# Autodesk Inventor assembly: CNC-FullAssembly
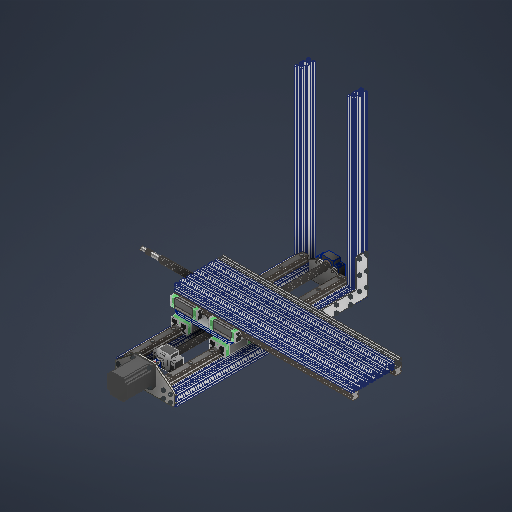
[picture p0: Inventor's stored thumbnail of the model, 512x512]
Saved by Autodesk Inventor 2026.2 (Build 302298000, 298)
## iProperties
Created: 2026-06-14
Part Number: CNC-FullAssembly
Document SubType Name: Assembly
Designer: Kenji
Mass: 13300 g
Surface Area: 16623.1 cm^2
Volume: 2793.26 cm^3
Density: 4.76145 g/cm^3
Author: Kenji
## Documents named in this file (29)
- C:\Users\Kenji\Documents\GitHub\DiyCNC-\CNC-FullAssembly.iam
- C:\Users\Kenji\Documents\GitHub\DiyCNC-\COTS-Parts\40x40x500mm-Extrusion.ipt
- C:\Users\Kenji\Documents\GitHub\DiyCNC-\COTS-Parts\SFU1605-BallScrewNut.iam
- C:\Users\Kenji\Documents\GitHub\DiyCNC-\COTS-Parts\DSG16H-BallScrewFixtureBlock.ipt
- C:\Users\Kenji\Documents\GitHub\DiyCNC-\COTS-Parts\SFU1605-BallScrew500mm.ipt
- C:\Users\Kenji\Documents\GitHub\DiyCNC-\COTS-Parts\BK12-BallScrewStabilizer.iam
- C:\Users\Kenji\Documents\GitHub\DiyCNC-\COTS-Parts\HGR20R-LinearRail500mm.ipt
- C:\Users\Kenji\Documents\GitHub\DiyCNC-\COTS-Parts\HGH20-LinearRailCarriage.iam
- C:\Users\Kenji\Documents\GitHub\DiyCNC-\COTS-Parts\91274A131_M5x20mm.ipt
- C:\Users\Kenji\Documents\GitHub\DiyCNC-\COTS-Parts\91290A231-M5x15mm.ipt
- C:\Users\Kenji\Documents\GitHub\DiyCNC-\COTS-Parts\Nema23-StepperMotor.ipt
- C:\Users\Kenji\Documents\GitHub\DiyCNC-\COTS-Parts\MH2025-6.35x10mmCoupler.iam
- C:\Users\Kenji\Documents\GitHub\DiyCNC-\COTS-Parts\BF12-BallScrewStabilizer2.ipt
- C:\Users\Kenji\Documents\GitHub\DiyCNC-\CNC-000-StructureGusset1.ipt
- C:\Users\Kenji\Documents\GitHub\DiyCNC-\COTS-Parts\20x40x500mm-Extrusion.ipt
- C:\Users\Kenji\Documents\GitHub\DiyCNC-\CNC-001-StructureGusset2.ipt
- C:\Users\Kenji\Documents\GitHub\DiyCNC-\CNC-002-ShimStructureGusset2.ipt
- C:\Users\Kenji\Documents\GitHub\DiyCNC-\COTS-Parts\90576A104-M5-NylockNut.ipt
- C:\Users\Kenji\Documents\GitHub\DiyCNC-\COTS-Parts\91292A195-M5x45mm.ipt
- C:\Users\Kenji\Documents\GitHub\DiyCNC-\CNC-003-StructureGusset3.ipt
- C:\Users\Kenji\Documents\GitHub\DiyCNC-\CNC-004-Nema23Shim.ipt
- C:\Users\Kenji\Documents\GitHub\DiyCNC-\COTS-Parts\91274A125-M5x8mm.ipt
- C:\Users\Kenji\Documents\GitHub\DiyCNC-\CNC-005-XAxisMount1.ipt
- C:\Users\Kenji\Documents\GitHub\DiyCNC-\COTS-Parts\91263A832-M5x10mm-Countersink.ipt
- C:\Users\Kenji\Documents\GitHub\DiyCNC-\CNC-006-XAxisMount2.ipt
- C:\Users\Kenji\Documents\GitHub\DiyCNC-\COTS-Parts\92095A495-M8-18mm-ButtonHead.ipt
- C:\Users\Kenji\Documents\GitHub\DiyCNC-\COTS-Parts\94645A210-M8-NylockNut.ipt
- C:\Users\Kenji\Documents\GitHub\DiyCNC-\COTS-Parts\20x40x500mm-Extrusion2.ipt
- C:\Users\Kenji\Documents\GitHub\DiyCNC-\COTS-Parts\20x20x500mm_Extrusion.ipt
## Components (172 placed, 28 different names)
1. 40x40x500mm-Extrusion:1 — Mate:1, Mate:2, Flush:1, Flush:2, Flush:3, Angle:1, Mate:6, Mate:12, Flush:5, Flush:6, Angle:3, Angle:4, Mate:46, Flush:20, Flush:21, Mate:48, Mate:49, Mate:50, Flush:35
2. 40x40x500mm-Extrusion:2 — Flush:2, Flush:3, Mate:7, Angle:2, Mate:11, Flush:9, Mate:39, Mate:40, Mate:41, Flush:22, Mate:47, Flush:23, Flush:38
3. SFU1605-BallScrewNut:1 [sub-assembly] — Mate:3, Mate:4, Mate:5, Mate:8, Mate:21, Mate:22, Mate:23, Mate:24, Mate:25, Mate:26, Mate:27
4. DSG16H-BallScrewFixtureBlock:1 — Mate:3, Mate:4, Mate:5, Angle:1, Mate:6, Mate:7, Flush:14, Mate:20, Rotation/Translation:2, Angle:6, Mate:98, Mate:99
5. SFU1605-BallScrew500mm:1 — Mate:8, Mate:9, Mate:10, Mate:30, Mate:34, Mate:35, Mate:36, Rotation/Translation:2
6. BK12-BallScrewStabilizer:1 [sub-assembly] — Mate:9, Mate:10, Angle:2
7. HGR20R-LinearRail500mm:1 — Mate:12, Flush:5, Flush:6, Flush:7, Flush:8, Mate:13, Mate:14, Mate:17, Mate:28, Mate:29, Mate:37
8. HGR20R-LinearRail500mm:2 — Mate:11, Flush:7, Flush:8, Flush:9, Mate:15, Mate:16, Mate:19
9. HGH20-LinearRailCarriage:1 [sub-assembly] — Mate:13, Mate:14, Flush:10, Flush:11, Mate:18, Flush:14, Mate:100
10. HGH20-LinearRailCarriage:2 [sub-assembly] — Mate:19, Flush:12, Flush:13
11. HGH20-LinearRailCarriage:3 [sub-assembly] — Mate:15, Mate:16, Flush:10, Flush:12, Mate:20
12. HGH20-LinearRailCarriage:4 [sub-assembly] — Mate:17, Flush:11, Mate:18, Flush:13
13. 91274A131_M5x20mm:1 — Mate:21, Mate:22, Flush:17, Flush:18
14. 91274A131_M5x20mm:2 — Mate:26, Flush:15, Flush:16
15. 91274A131_M5x20mm:3 — Mate:27, Flush:15
16. 91274A131_M5x20mm:4 — Mate:25, Flush:16, Flush:17
17. 91274A131_M5x20mm:5 — Mate:23, Flush:18, Flush:19
18. 91274A131_M5x20mm:6 — Mate:24, Flush:19
19. Nema23-StepperMotor:1 — Mate:32, Angle:3, Mate:33, Mate:59, Mate:60, Mate:61, Mate:62, Mate:63
20. MH2025-6.35x10mmCoupler:1 [sub-assembly] — Mate:30, Mate:32, Mate:33, Mate:34
21. BF12-BallScrewStabilizer2:1 — Mate:35, Mate:36, Angle:4, Mate:37, Mate:56, Mate:57, Mate:58
22. CNC-000-StructureGusset1:1 — Mate:39, Mate:40, Mate:41, Mate:42, Mate:43, Mate:44, Mate:45, Mate:65, Mate:77, Mate:79
23. 20x40x500mm-Extrusion:1 — Mate:46, Flush:20, Flush:21, Mate:71, Mate:72, Mate:73, Mate:74, Mate:75, Flush:36
24. 20x40x500mm-Extrusion:2 — Flush:22, Mate:47, Flush:23, Mate:69, Mate:70, Mate:76, Flush:37
25. CNC-001-StructureGusset2:1 — Mate:48, Mate:49, Mate:50, Mate:51, Mate:52, Mate:53, Mate:54, Mate:55
26. 91290A231-M5x15mm:27 — Mate:51, Mate:52, Flush:25, Flush:26
27. 91290A231-M5x15mm:28 — Mate:54, Flush:24, Flush:25
28. 91290A231-M5x15mm:29 — Mate:55, Flush:24
29. 91290A231-M5x15mm:30 — Mate:53, Flush:26
30. CNC-002-ShimStructureGusset2:1 — Mate:56, Mate:57, Mate:58
31. 91274A131_M5x20mm:7 — Mate:60, Flush:29, Mate:67
32. 91274A131_M5x20mm:8 — Mate:62, Mate:63, Flush:27, Mate:68
33. 91274A131_M5x20mm:9 — Mate:59, Flush:28, Flush:29, Mate:64
34. 91274A131_M5x20mm:10 — Mate:61, Flush:27, Flush:28, Mate:66
35. 90576A104-M5-NylockNut:1 — Mate:64, Mate:65, Flush:32
36. 90576A104-M5-NylockNut:2 — Mate:66, Flush:30, Mate:78
37. 90576A104-M5-NylockNut:3 — Mate:68, Flush:30, Flush:31
38. 90576A104-M5-NylockNut:4 — Mate:67, Flush:31, Flush:32
39. 91292A195-M5x45mm:1 — Mate:69, Flush:33, Flush:34
40. 91292A195-M5x45mm:2 — Mate:70, Flush:34
41. 91292A195-M5x45mm:3 — Mate:72, Mate:73
42. 91292A195-M5x45mm:4 — Mate:71, Mate:74, Flush:33
43. CNC-003-StructureGusset3:1 — Mate:75, Flush:35, Flush:36, Mate:80, Mate:81, Mate:82, Mate:83
44. CNC-003-StructureGusset3:2 — Mate:76, Flush:37, Flush:38, Mate:84, Mate:85, Mate:86, Mate:87
45. CNC-004-Nema23Shim:1 — Mate:77, Mate:78, Mate:79
46. HGH20-LinearRailCarriage:5 [sub-assembly] — Mate:91, Mate:92, Mate:131, Mate:132, Mate:133
47. HGH20-LinearRailCarriage:6 [sub-assembly] — Mate:128, Mate:129, Mate:130
48. HGH20-LinearRailCarriage:7 [sub-assembly] — Mate:125, Mate:126, Mate:127
49. HGH20-LinearRailCarriage:8 [sub-assembly] — Mate:134, Mate:135, Mate:136, Mate:137, Mate:138
50. HGR20R-LinearRail500mm:3 — Flush:50, Mate:137, Mate:138
51. HGR20R-LinearRail500mm:4 — Mate:91, Mate:92, Flush:50, Mate:192, Flush:106, Flush:107
52. DSG16H-BallScrewFixtureBlock:2 — Angle:6, Mate:94, Mate:95, Mate:96, Mate:97, Mate:121, Mate:122, Mate:123
53. SFU1605-BallScrewNut:2 [sub-assembly] — Mate:94, Mate:95, Mate:96, Mate:139, Mate:140, Mate:141, Mate:142, Mate:143, Mate:144, Mate:145
54. SFU1605-BallScrew500mm:2 — Mate:97
55. CNC-005-XAxisMount1:1 — Mate:98, Mate:99, Mate:100, Mate:101, Flush:53, Mate:102, Mate:103, Mate:104, Mate:105, Mate:106, Mate:107, Mate:108, Flush:57, Flush:58, Flush:59, Flush:60, Mate:109, Mate:110, Mate:111, Mate:112, Flush:61, Flush:63, Mate:113, Mate:114, Mate:115, Mate:116, Flush:65, Flush:66, Flush:67, Flush:68, Mate:117, Mate:118, Mate:119, Mate:120, Flush:69, Flush:70, Flush:71, Flush:72, Mate:124, Angle:7, Mate:166, Mate:177, Mate:179, Mate:181, Mate:183, Mate:186, Mate:187, Mate:190, Mate:191
56. 91263A832-M5x10mm-Countersink:1 — Mate:101, Flush:53, Flush:56
57. 91263A832-M5x10mm-Countersink:2 — Mate:104, Flush:55
58. 91263A832-M5x10mm-Countersink:3 — Mate:102, Flush:54, Flush:55, Flush:56
59. 91263A832-M5x10mm-Countersink:4 — Mate:103, Flush:54
60. 91263A832-M5x10mm-Countersink:5 — Mate:105, Flush:59
61. 91263A832-M5x10mm-Countersink:6 — Mate:106, Flush:58
62. 91263A832-M5x10mm-Countersink:7 — Mate:108, Flush:57
63. 91263A832-M5x10mm-Countersink:8 — Mate:107, Flush:60
64. 91263A832-M5x10mm-Countersink:9 — Mate:112, Flush:62
65. 91263A832-M5x10mm-Countersink:10 — Mate:111, Flush:61, Flush:62
66. 91263A832-M5x10mm-Countersink:11 — Mate:109, Flush:63, Flush:64
67. 91263A832-M5x10mm-Countersink:12 — Mate:110, Flush:64
68. 91263A832-M5x10mm-Countersink:13 — Mate:113, Flush:65
69. 91263A832-M5x10mm-Countersink:14 — Mate:116, Flush:67
70. 91263A832-M5x10mm-Countersink:15 — Mate:115, Flush:66
71. 91263A832-M5x10mm-Countersink:16 — Mate:114, Flush:68
72. 91263A832-M5x10mm-Countersink:17 — Mate:118, Flush:71
73. 91263A832-M5x10mm-Countersink:18 — Mate:119, Flush:69
74. 91263A832-M5x10mm-Countersink:19 — Mate:117, Flush:72
75. 91263A832-M5x10mm-Countersink:20 — Mate:120, Flush:70
76. CNC-006-XAxisMount2:1 — Mate:121, Mate:122, Mate:123, Mate:124, Angle:7, Mate:125, Mate:126, Mate:127, Mate:128, Mate:129, Mate:130, Mate:131, Mate:132, Mate:133, Mate:134, Mate:135, Mate:136, Mate:146, Mate:147, Mate:148, Mate:149, Flush:78, Flush:79, Flush:81, Mate:150, Mate:151, Mate:152, Mate:153, Flush:82, Flush:83, Flush:84, Flush:85, Mate:154, Mate:155, Mate:156, Mate:157, Flush:86, Flush:87, Mate:158, Mate:159, Mate:160, Mate:161, Flush:90, Flush:91, Flush:92, Flush:93, Mate:162, Mate:163, Mate:164, Mate:165, Flush:94, Flush:95, Flush:96, Flush:97, Mate:166, Mate:167, Mate:168, Mate:169, Mate:170, Mate:171, Mate:172, Mate:173, Mate:174, Mate:175
77. 91274A131_M5x20mm:11 — Mate:139, Mate:140, Flush:74, Flush:75
78. 91274A131_M5x20mm:12 — Mate:145, Flush:76, Flush:77
79. 91274A131_M5x20mm:13 — Mate:144, Flush:77
80. 91274A131_M5x20mm:14 — Mate:141, Flush:73, Flush:74
81. 91274A131_M5x20mm:15 — Mate:143, Flush:75
82. 91274A131_M5x20mm:16 — Mate:142, Flush:73, Flush:76
83. 91263A832-M5x10mm-Countersink:21 — Mate:149, Flush:78
84. 91263A832-M5x10mm-Countersink:22 — Mate:146, Flush:80
85. 91263A832-M5x10mm-Countersink:23 — Mate:147, Flush:79, Flush:80
86. 91263A832-M5x10mm-Countersink:24 — Mate:148, Flush:81
87. 91263A832-M5x10mm-Countersink:25 — Mate:150, Flush:85
88. 91263A832-M5x10mm-Countersink:26 — Mate:153, Flush:83
89. 91263A832-M5x10mm-Countersink:27 — Mate:151, Flush:82
90. 91263A832-M5x10mm-Countersink:28 — Mate:152, Flush:84
91. 91263A832-M5x10mm-Countersink:29 — Mate:156, Flush:87, Flush:88
92. 91263A832-M5x10mm-Countersink:30 — Mate:155, Flush:89
93. 91263A832-M5x10mm-Countersink:31 — Mate:154, Flush:88, Flush:89
94. 91263A832-M5x10mm-Countersink:32 — Mate:157, Flush:86
95. 91263A832-M5x10mm-Countersink:33 — Mate:159, Flush:93
96. 91263A832-M5x10mm-Countersink:34 — Mate:160, Flush:91
97. 91263A832-M5x10mm-Countersink:35 — Mate:158, Flush:92
98. 91263A832-M5x10mm-Countersink:36 — Mate:161, Flush:90
99. 91263A832-M5x10mm-Countersink:37 — Mate:164, Flush:95
100. 91263A832-M5x10mm-Countersink:38 — Mate:162, Flush:96
101. 91263A832-M5x10mm-Countersink:39 — Mate:163, Flush:97
102. 91263A832-M5x10mm-Countersink:40 — Mate:165, Flush:94
103. 92095A495-M8-18mm-ButtonHead:1 — Mate:167, Flush:98, Flush:99, Flush:102, Mate:176
104. 92095A495-M8-18mm-ButtonHead:2 — Mate:168, Flush:99, Flush:104, Mate:178
105. 92095A495-M8-18mm-ButtonHead:3 — Mate:169, Mate:170, Flush:98, Flush:100, Mate:180
106. 92095A495-M8-18mm-ButtonHead:8 — Mate:171, Flush:100, Mate:182
107. 92095A495-M8-18mm-ButtonHead:9 — Mate:174, Flush:103, Flush:104, Mate:188
108. 92095A495-M8-18mm-ButtonHead:10 — Mate:175, Flush:103, Mate:189
109. 92095A495-M8-18mm-ButtonHead:11 — Mate:172, Flush:101, Flush:102, Mate:184
110. 92095A495-M8-18mm-ButtonHead:12 — Mate:173, Flush:101, Mate:185
111. 94645A210-M8-NylockNut:1 — Mate:176, Mate:177
112. 94645A210-M8-NylockNut:2 — Mate:178, Mate:179
113. 94645A210-M8-NylockNut:3 — Mate:180, Mate:181
114. 94645A210-M8-NylockNut:4 — Mate:182, Mate:183
115. 94645A210-M8-NylockNut:5 — Mate:184, Mate:187
116. 94645A210-M8-NylockNut:6 — Mate:185, Mate:186
117. 94645A210-M8-NylockNut:7 — Mate:188, Mate:191
118. 94645A210-M8-NylockNut:8 — Mate:189, Mate:190
119. 20x40x500mm-Extrusion2:1 — Mate:192, Flush:106, Flush:107, Flush:108, Mate:193, Flush:109
120. 20x40x500mm-Extrusion2:2 — Flush:108, Mate:193, Flush:109, Flush:110, Flush:111, Mate:194
121. 20x40x500mm-Extrusion2:3 — Flush:110, Flush:111, Mate:194, Flush:112, Flush:113, Mate:195
122. 20x20x500mm_Extrusion:1 — Flush:112, Flush:113, Mate:195
123. 91290A231-M5x15mm:1 — Mate:28, Mate:29
124. 91290A231-M5x15mm:2
125. 91290A231-M5x15mm:3
126. 91290A231-M5x15mm:4
127. 91290A231-M5x15mm:5
128. 91290A231-M5x15mm:6
129. 91290A231-M5x15mm:7
130. 91290A231-M5x15mm:8
131. 91290A231-M5x15mm:9
132. 91290A231-M5x15mm:10
133. 91290A231-M5x15mm:11
134. 91290A231-M5x15mm:12
135. 91290A231-M5x15mm:13
136. 91290A231-M5x15mm:14
137. 91290A231-M5x15mm:15
138. 91290A231-M5x15mm:16
139. 91290A231-M5x15mm:17
140. 91290A231-M5x15mm:18
141. 91290A231-M5x15mm:20 — Mate:44, Mate:45
142. 91290A231-M5x15mm:21
143. 91290A231-M5x15mm:22
144. 91290A231-M5x15mm:23
145. 91290A231-M5x15mm:19 — Mate:42, Mate:43
146. 91290A231-M5x15mm:24
147. 91290A231-M5x15mm:25
148. 91290A231-M5x15mm:26
149. 91274A125-M5x8mm:1 — Mate:80, Mate:81
150. 91274A125-M5x8mm:2
151. 91274A125-M5x8mm:3
152. 91274A125-M5x8mm:4
153. 91274A125-M5x8mm:5
154. 91274A125-M5x8mm:6
155. 91274A125-M5x8mm:7 — Mate:82, Mate:83
156. 91274A125-M5x8mm:8
157. 91274A125-M5x8mm:9
158. 91274A125-M5x8mm:10
159. 91274A125-M5x8mm:11
160. 91274A125-M5x8mm:12
161. 91274A125-M5x8mm:13 — Mate:84, Mate:85
162. 91274A125-M5x8mm:14
163. 91274A125-M5x8mm:15
164. 91274A125-M5x8mm:16
165. 91274A125-M5x8mm:17
166. 91274A125-M5x8mm:18
167. 91274A125-M5x8mm:19 — Mate:86, Mate:87
168. 91274A125-M5x8mm:20
169. 91274A125-M5x8mm:21
170. 91274A125-M5x8mm:22
171. 91274A125-M5x8mm:23
172. 91274A125-M5x8mm:24
## Component patterns: (18 elements, first: 91290A231-M5x15mm:1), (4 elements, first: 91290A231-M5x15mm:20), (4 elements, first: 91290A231-M5x15mm:19), (6 elements, first: 91274A125-M5x8mm:1), (6 elements, first: 91274A125-M5x8mm:7), (6 elements, first: 91274A125-M5x8mm:13), (6 elements, first: 91274A125-M5x8mm:19)
## Relationships (294: Mate 189, Flush 98, Angle 6, RelateRotateTranslate 1)
- Mate:1 (-20 mm): 40x40x500mm-Extrusion:1
- Mate:2 (-20 mm): 40x40x500mm-Extrusion:1
- Flush:1 (-250 mm): 40x40x500mm-Extrusion:1
- Flush:2: 40x40x500mm-Extrusion:1 ↔ 40x40x500mm-Extrusion:2
- Flush:3: 40x40x500mm-Extrusion:1 ↔ 40x40x500mm-Extrusion:2
- Mate:3: SFU1605-BallScrewNut:1 ↔ DSG16H-BallScrewFixtureBlock:1
- Mate:4: SFU1605-BallScrewNut:1 ↔ DSG16H-BallScrewFixtureBlock:1
- Mate:5: SFU1605-BallScrewNut:1 ↔ DSG16H-BallScrewFixtureBlock:1
- Angle:1 (0 deg): 40x40x500mm-Extrusion:1 ↔ DSG16H-BallScrewFixtureBlock:1
- Mate:6 (18 mm): 40x40x500mm-Extrusion:1 ↔ DSG16H-BallScrewFixtureBlock:1
- Mate:7 (18 mm): 40x40x500mm-Extrusion:2 ↔ DSG16H-BallScrewFixtureBlock:1
- Mate:8: SFU1605-BallScrewNut:1 ↔ SFU1605-BallScrew500mm:1
- Mate:9: SFU1605-BallScrew500mm:1 ↔ BK12-BallScrewStabilizer:1
- Mate:10: SFU1605-BallScrew500mm:1 ↔ BK12-BallScrewStabilizer:1
- Angle:2 (0 deg): 40x40x500mm-Extrusion:2 ↔ BK12-BallScrewStabilizer:1
- Mate:11: 40x40x500mm-Extrusion:2 ↔ HGR20R-LinearRail500mm:2
- Mate:12: 40x40x500mm-Extrusion:1 ↔ HGR20R-LinearRail500mm:1
- Flush:5: 40x40x500mm-Extrusion:1 ↔ HGR20R-LinearRail500mm:1
- Flush:6: 40x40x500mm-Extrusion:1 ↔ HGR20R-LinearRail500mm:1
- Flush:7: HGR20R-LinearRail500mm:1 ↔ HGR20R-LinearRail500mm:2
- Flush:8: HGR20R-LinearRail500mm:1 ↔ HGR20R-LinearRail500mm:2
- Flush:9: 40x40x500mm-Extrusion:2 ↔ HGR20R-LinearRail500mm:2
- Mate:13: HGR20R-LinearRail500mm:1 ↔ HGH20-LinearRailCarriage:1
- Mate:14: HGR20R-LinearRail500mm:1 ↔ HGH20-LinearRailCarriage:1
- Mate:15: HGR20R-LinearRail500mm:2 ↔ HGH20-LinearRailCarriage:3
- Mate:16: HGR20R-LinearRail500mm:2 ↔ HGH20-LinearRailCarriage:3
- Flush:10: HGH20-LinearRailCarriage:1 ↔ HGH20-LinearRailCarriage:3
- Mate:17: HGR20R-LinearRail500mm:1 ↔ HGH20-LinearRailCarriage:4
- Flush:11: HGH20-LinearRailCarriage:1 ↔ HGH20-LinearRailCarriage:4
- Mate:18 (40 mm): HGH20-LinearRailCarriage:1 ↔ HGH20-LinearRailCarriage:4
- Mate:19: HGR20R-LinearRail500mm:2 ↔ HGH20-LinearRailCarriage:2
- Flush:12: HGH20-LinearRailCarriage:2 ↔ HGH20-LinearRailCarriage:3
- Flush:13: HGH20-LinearRailCarriage:2 ↔ HGH20-LinearRailCarriage:4
- Flush:14: DSG16H-BallScrewFixtureBlock:1 ↔ HGH20-LinearRailCarriage:1
- Mate:20: DSG16H-BallScrewFixtureBlock:1 ↔ HGH20-LinearRailCarriage:3
- Mate:21: SFU1605-BallScrewNut:1 ↔ 91274A131_M5x20mm:1
- Mate:22: SFU1605-BallScrewNut:1 ↔ 91274A131_M5x20mm:1
- Mate:23: SFU1605-BallScrewNut:1 ↔ 91274A131_M5x20mm:5
- Mate:24: SFU1605-BallScrewNut:1 ↔ 91274A131_M5x20mm:6
- Mate:25: SFU1605-BallScrewNut:1 ↔ 91274A131_M5x20mm:4
- Mate:26: SFU1605-BallScrewNut:1 ↔ 91274A131_M5x20mm:2
- Mate:27: SFU1605-BallScrewNut:1 ↔ 91274A131_M5x20mm:3
- Flush:15: 91274A131_M5x20mm:2 ↔ 91274A131_M5x20mm:3
- Flush:16: 91274A131_M5x20mm:2 ↔ 91274A131_M5x20mm:4
- Flush:17: 91274A131_M5x20mm:1 ↔ 91274A131_M5x20mm:4
- Flush:18: 91274A131_M5x20mm:1 ↔ 91274A131_M5x20mm:5
- Flush:19: 91274A131_M5x20mm:5 ↔ 91274A131_M5x20mm:6
- Mate:28: HGR20R-LinearRail500mm:1 ↔ 91290A231-M5x15mm:1
- Mate:29: HGR20R-LinearRail500mm:1 ↔ 91290A231-M5x15mm:1
- Mate:30: SFU1605-BallScrew500mm:1 ↔ MH2025-6.35x10mmCoupler:1
- Mate:32: Nema23-StepperMotor:1 ↔ MH2025-6.35x10mmCoupler:1
- Angle:3 (0 deg): 40x40x500mm-Extrusion:1 ↔ Nema23-StepperMotor:1
- Mate:33 (2 mm): Nema23-StepperMotor:1 ↔ MH2025-6.35x10mmCoupler:1
- Mate:34 (2 mm): SFU1605-BallScrew500mm:1 ↔ MH2025-6.35x10mmCoupler:1
- Mate:35: SFU1605-BallScrew500mm:1 ↔ BF12-BallScrewStabilizer2:1
- Mate:36: SFU1605-BallScrew500mm:1 ↔ BF12-BallScrewStabilizer2:1
- Angle:4 (0 deg): 40x40x500mm-Extrusion:1 ↔ BF12-BallScrewStabilizer2:1
- Mate:37 (9.525 mm): HGR20R-LinearRail500mm:1 ↔ BF12-BallScrewStabilizer2:1
- Mate:39: 40x40x500mm-Extrusion:2 ↔ CNC-000-StructureGusset1:1
- Mate:40: 40x40x500mm-Extrusion:2 ↔ CNC-000-StructureGusset1:1
- Mate:41: 40x40x500mm-Extrusion:2 ↔ CNC-000-StructureGusset1:1
- Mate:42: CNC-000-StructureGusset1:1 ↔ 91290A231-M5x15mm:19
- Mate:43: CNC-000-StructureGusset1:1 ↔ 91290A231-M5x15mm:19
- Mate:44: CNC-000-StructureGusset1:1 ↔ 91290A231-M5x15mm:20
- Mate:45: CNC-000-StructureGusset1:1 ↔ 91290A231-M5x15mm:20
- Mate:46: 40x40x500mm-Extrusion:1 ↔ 20x40x500mm-Extrusion:1
- Flush:20: 40x40x500mm-Extrusion:1 ↔ 20x40x500mm-Extrusion:1
- Flush:21: 40x40x500mm-Extrusion:1 ↔ 20x40x500mm-Extrusion:1
- Flush:22: 40x40x500mm-Extrusion:2 ↔ 20x40x500mm-Extrusion:2
- Mate:47: 40x40x500mm-Extrusion:2 ↔ 20x40x500mm-Extrusion:2
- Flush:23: 40x40x500mm-Extrusion:2 ↔ 20x40x500mm-Extrusion:2
- Mate:48: 40x40x500mm-Extrusion:1 ↔ CNC-001-StructureGusset2:1
- Mate:49: 40x40x500mm-Extrusion:1 ↔ CNC-001-StructureGusset2:1
- Mate:50: 40x40x500mm-Extrusion:1 ↔ CNC-001-StructureGusset2:1
- Mate:51: CNC-001-StructureGusset2:1 ↔ 91290A231-M5x15mm:27
- Mate:52: CNC-001-StructureGusset2:1 ↔ 91290A231-M5x15mm:27
- Mate:53: CNC-001-StructureGusset2:1 ↔ 91290A231-M5x15mm:30
- Mate:54: CNC-001-StructureGusset2:1 ↔ 91290A231-M5x15mm:28
- Mate:55: CNC-001-StructureGusset2:1 ↔ 91290A231-M5x15mm:29
- Flush:24: 91290A231-M5x15mm:28 ↔ 91290A231-M5x15mm:29
- Flush:25: 91290A231-M5x15mm:27 ↔ 91290A231-M5x15mm:28
- Flush:26: 91290A231-M5x15mm:27 ↔ 91290A231-M5x15mm:30
- Mate:56: BF12-BallScrewStabilizer2:1 ↔ CNC-002-ShimStructureGusset2:1
- Mate:57: BF12-BallScrewStabilizer2:1 ↔ CNC-002-ShimStructureGusset2:1
- Mate:58: BF12-BallScrewStabilizer2:1 ↔ CNC-002-ShimStructureGusset2:1
- Mate:59: Nema23-StepperMotor:1 ↔ 91274A131_M5x20mm:9
- Mate:60: Nema23-StepperMotor:1 ↔ 91274A131_M5x20mm:7
- Mate:61: Nema23-StepperMotor:1 ↔ 91274A131_M5x20mm:10
- Mate:62: Nema23-StepperMotor:1 ↔ 91274A131_M5x20mm:8
- Mate:63: Nema23-StepperMotor:1 ↔ 91274A131_M5x20mm:8
- Flush:27: 91274A131_M5x20mm:8 ↔ 91274A131_M5x20mm:10
- Flush:28: 91274A131_M5x20mm:9 ↔ 91274A131_M5x20mm:10
- Flush:29: 91274A131_M5x20mm:7 ↔ 91274A131_M5x20mm:9
- Mate:64: 91274A131_M5x20mm:9 ↔ 90576A104-M5-NylockNut:1
- Mate:65: CNC-000-StructureGusset1:1 ↔ 90576A104-M5-NylockNut:1
- Mate:66: 91274A131_M5x20mm:10 ↔ 90576A104-M5-NylockNut:2
- Mate:67: 91274A131_M5x20mm:7 ↔ 90576A104-M5-NylockNut:4
- Mate:68: 91274A131_M5x20mm:8 ↔ 90576A104-M5-NylockNut:3
- Flush:30: 90576A104-M5-NylockNut:2 ↔ 90576A104-M5-NylockNut:3
- Flush:31: 90576A104-M5-NylockNut:3 ↔ 90576A104-M5-NylockNut:4
- Flush:32: 90576A104-M5-NylockNut:1 ↔ 90576A104-M5-NylockNut:4
- Mate:69: 20x40x500mm-Extrusion:2 ↔ 91292A195-M5x45mm:1
- Mate:70: 20x40x500mm-Extrusion:2 ↔ 91292A195-M5x45mm:2
- Mate:71: 20x40x500mm-Extrusion:1 ↔ 91292A195-M5x45mm:4
- Mate:72: 20x40x500mm-Extrusion:1 ↔ 91292A195-M5x45mm:3
- Mate:73: 20x40x500mm-Extrusion:1 ↔ 91292A195-M5x45mm:3
- Mate:74: 20x40x500mm-Extrusion:1 ↔ 91292A195-M5x45mm:4
- Flush:33: 91292A195-M5x45mm:1 ↔ 91292A195-M5x45mm:4
- Flush:34: 91292A195-M5x45mm:1 ↔ 91292A195-M5x45mm:2
- Mate:75: 20x40x500mm-Extrusion:1 ↔ CNC-003-StructureGusset3:1
- Flush:35 (4.225 mm): 40x40x500mm-Extrusion:1 ↔ CNC-003-StructureGusset3:1
- Flush:36 (-4.225 mm): 20x40x500mm-Extrusion:1 ↔ CNC-003-StructureGusset3:1
- Mate:76: 20x40x500mm-Extrusion:2 ↔ CNC-003-StructureGusset3:2
- Flush:37 (-4.225 mm): 20x40x500mm-Extrusion:2 ↔ CNC-003-StructureGusset3:2
- Flush:38 (4.225 mm): 40x40x500mm-Extrusion:2 ↔ CNC-003-StructureGusset3:2
- Mate:77: CNC-000-StructureGusset1:1 ↔ CNC-004-Nema23Shim:1
- Mate:78: 90576A104-M5-NylockNut:2 ↔ CNC-004-Nema23Shim:1
- Mate:79: CNC-000-StructureGusset1:1 ↔ CNC-004-Nema23Shim:1
- Rotation/Translation:2 [RelateRotateTranslate] (5 mm): DSG16H-BallScrewFixtureBlock:1 ↔ SFU1605-BallScrew500mm:1
- Mate:80: CNC-003-StructureGusset3:1 ↔ 91274A125-M5x8mm:1
- Mate:81: CNC-003-StructureGusset3:1 ↔ 91274A125-M5x8mm:1
- Mate:82: CNC-003-StructureGusset3:1 ↔ 91274A125-M5x8mm:7
- Mate:83: CNC-003-StructureGusset3:1 ↔ 91274A125-M5x8mm:7
- Mate:84: CNC-003-StructureGusset3:2 ↔ 91274A125-M5x8mm:13
- Mate:85: CNC-003-StructureGusset3:2 ↔ 91274A125-M5x8mm:13
- Mate:86: CNC-003-StructureGusset3:2 ↔ 91274A125-M5x8mm:19
- Mate:87: CNC-003-StructureGusset3:2 ↔ 91274A125-M5x8mm:19
- Mate:91: HGH20-LinearRailCarriage:5 ↔ HGR20R-LinearRail500mm:4
- Mate:92: HGH20-LinearRailCarriage:5 ↔ HGR20R-LinearRail500mm:4
- Flush:50: HGR20R-LinearRail500mm:3 ↔ HGR20R-LinearRail500mm:4
- Angle:6 (180 deg): DSG16H-BallScrewFixtureBlock:1 ↔ DSG16H-BallScrewFixtureBlock:2
- Mate:94: DSG16H-BallScrewFixtureBlock:2 ↔ SFU1605-BallScrewNut:2
- Mate:95: DSG16H-BallScrewFixtureBlock:2 ↔ SFU1605-BallScrewNut:2
- Mate:96: DSG16H-BallScrewFixtureBlock:2 ↔ SFU1605-BallScrewNut:2
- Mate:97: DSG16H-BallScrewFixtureBlock:2 ↔ SFU1605-BallScrew500mm:2
- Mate:98: DSG16H-BallScrewFixtureBlock:1 ↔ CNC-005-XAxisMount1:1
- Mate:99: DSG16H-BallScrewFixtureBlock:1 ↔ CNC-005-XAxisMount1:1
- Mate:100: HGH20-LinearRailCarriage:1 ↔ CNC-005-XAxisMount1:1
- Mate:101: CNC-005-XAxisMount1:1 ↔ 91263A832-M5x10mm-Countersink:1
- Flush:53: CNC-005-XAxisMount1:1 ↔ 91263A832-M5x10mm-Countersink:1
- Mate:102: CNC-005-XAxisMount1:1 ↔ 91263A832-M5x10mm-Countersink:3
- Mate:103: CNC-005-XAxisMount1:1 ↔ 91263A832-M5x10mm-Countersink:4
- Mate:104: CNC-005-XAxisMount1:1 ↔ 91263A832-M5x10mm-Countersink:2
- Flush:54: 91263A832-M5x10mm-Countersink:3 ↔ 91263A832-M5x10mm-Countersink:4
- Flush:55: 91263A832-M5x10mm-Countersink:2 ↔ 91263A832-M5x10mm-Countersink:3
- Flush:56: 91263A832-M5x10mm-Countersink:1 ↔ 91263A832-M5x10mm-Countersink:3
- Mate:105: CNC-005-XAxisMount1:1 ↔ 91263A832-M5x10mm-Countersink:5
- Mate:106: CNC-005-XAxisMount1:1 ↔ 91263A832-M5x10mm-Countersink:6
- Mate:107: CNC-005-XAxisMount1:1 ↔ 91263A832-M5x10mm-Countersink:8
- Mate:108: CNC-005-XAxisMount1:1 ↔ 91263A832-M5x10mm-Countersink:7
- Flush:57: CNC-005-XAxisMount1:1 ↔ 91263A832-M5x10mm-Countersink:7
- Flush:58: CNC-005-XAxisMount1:1 ↔ 91263A832-M5x10mm-Countersink:6
- Flush:59: CNC-005-XAxisMount1:1 ↔ 91263A832-M5x10mm-Countersink:5
- Flush:60: CNC-005-XAxisMount1:1 ↔ 91263A832-M5x10mm-Countersink:8
- Mate:109: CNC-005-XAxisMount1:1 ↔ 91263A832-M5x10mm-Countersink:11
- Mate:110: CNC-005-XAxisMount1:1 ↔ 91263A832-M5x10mm-Countersink:12
- Mate:111: CNC-005-XAxisMount1:1 ↔ 91263A832-M5x10mm-Countersink:10
- Mate:112: CNC-005-XAxisMount1:1 ↔ 91263A832-M5x10mm-Countersink:9
- Flush:61: CNC-005-XAxisMount1:1 ↔ 91263A832-M5x10mm-Countersink:10
- Flush:62: 91263A832-M5x10mm-Countersink:9 ↔ 91263A832-M5x10mm-Countersink:10
- Flush:63: CNC-005-XAxisMount1:1 ↔ 91263A832-M5x10mm-Countersink:11
- Flush:64: 91263A832-M5x10mm-Countersink:11 ↔ 91263A832-M5x10mm-Countersink:12
- Mate:113: CNC-005-XAxisMount1:1 ↔ 91263A832-M5x10mm-Countersink:13
- Mate:114: CNC-005-XAxisMount1:1 ↔ 91263A832-M5x10mm-Countersink:16
- Mate:115: CNC-005-XAxisMount1:1 ↔ 91263A832-M5x10mm-Countersink:15
- Mate:116: CNC-005-XAxisMount1:1 ↔ 91263A832-M5x10mm-Countersink:14
- Flush:65: CNC-005-XAxisMount1:1 ↔ 91263A832-M5x10mm-Countersink:13
- Flush:66: CNC-005-XAxisMount1:1 ↔ 91263A832-M5x10mm-Countersink:15
- Flush:67: CNC-005-XAxisMount1:1 ↔ 91263A832-M5x10mm-Countersink:14
- Flush:68: CNC-005-XAxisMount1:1 ↔ 91263A832-M5x10mm-Countersink:16
- Mate:117: CNC-005-XAxisMount1:1 ↔ 91263A832-M5x10mm-Countersink:19
- Mate:118: CNC-005-XAxisMount1:1 ↔ 91263A832-M5x10mm-Countersink:17
- Mate:119: CNC-005-XAxisMount1:1 ↔ 91263A832-M5x10mm-Countersink:18
- Mate:120: CNC-005-XAxisMount1:1 ↔ 91263A832-M5x10mm-Countersink:20
- Flush:69: CNC-005-XAxisMount1:1 ↔ 91263A832-M5x10mm-Countersink:18
- Flush:70: CNC-005-XAxisMount1:1 ↔ 91263A832-M5x10mm-Countersink:20
- Flush:71: CNC-005-XAxisMount1:1 ↔ 91263A832-M5x10mm-Countersink:17
- Flush:72: CNC-005-XAxisMount1:1 ↔ 91263A832-M5x10mm-Countersink:19
- Mate:121: DSG16H-BallScrewFixtureBlock:2 ↔ CNC-006-XAxisMount2:1
- Mate:122: DSG16H-BallScrewFixtureBlock:2 ↔ CNC-006-XAxisMount2:1
- Mate:123: DSG16H-BallScrewFixtureBlock:2 ↔ CNC-006-XAxisMount2:1
- Mate:124: CNC-005-XAxisMount1:1 ↔ CNC-006-XAxisMount2:1
- Angle:7 (0 deg): CNC-005-XAxisMount1:1 ↔ CNC-006-XAxisMount2:1
- Mate:125: HGH20-LinearRailCarriage:7 ↔ CNC-006-XAxisMount2:1
- Mate:126: HGH20-LinearRailCarriage:7 ↔ CNC-006-XAxisMount2:1
- Mate:127: HGH20-LinearRailCarriage:7 ↔ CNC-006-XAxisMount2:1
- Mate:128: HGH20-LinearRailCarriage:6 ↔ CNC-006-XAxisMount2:1
- Mate:129: HGH20-LinearRailCarriage:6 ↔ CNC-006-XAxisMount2:1
- Mate:130: HGH20-LinearRailCarriage:6 ↔ CNC-006-XAxisMount2:1
- Mate:131: HGH20-LinearRailCarriage:5 ↔ CNC-006-XAxisMount2:1
- Mate:132: HGH20-LinearRailCarriage:5 ↔ CNC-006-XAxisMount2:1
- Mate:133: HGH20-LinearRailCarriage:5 ↔ CNC-006-XAxisMount2:1
- Mate:134: HGH20-LinearRailCarriage:8 ↔ CNC-006-XAxisMount2:1
- Mate:135: HGH20-LinearRailCarriage:8 ↔ CNC-006-XAxisMount2:1
- Mate:136: HGH20-LinearRailCarriage:8 ↔ CNC-006-XAxisMount2:1
- Mate:137: HGH20-LinearRailCarriage:8 ↔ HGR20R-LinearRail500mm:3
- Mate:138: HGH20-LinearRailCarriage:8 ↔ HGR20R-LinearRail500mm:3
- Mate:139: SFU1605-BallScrewNut:2 ↔ 91274A131_M5x20mm:11
- Mate:140: SFU1605-BallScrewNut:2 ↔ 91274A131_M5x20mm:11
- Mate:141: SFU1605-BallScrewNut:2 ↔ 91274A131_M5x20mm:14
- Mate:142: SFU1605-BallScrewNut:2 ↔ 91274A131_M5x20mm:16
- Mate:143: SFU1605-BallScrewNut:2 ↔ 91274A131_M5x20mm:15
- Mate:144: SFU1605-BallScrewNut:2 ↔ 91274A131_M5x20mm:13
- Mate:145: SFU1605-BallScrewNut:2 ↔ 91274A131_M5x20mm:12
- Flush:73: 91274A131_M5x20mm:14 ↔ 91274A131_M5x20mm:16
- Flush:74: 91274A131_M5x20mm:11 ↔ 91274A131_M5x20mm:14
- Flush:75: 91274A131_M5x20mm:11 ↔ 91274A131_M5x20mm:15
- Flush:76: 91274A131_M5x20mm:12 ↔ 91274A131_M5x20mm:16
- Flush:77: 91274A131_M5x20mm:12 ↔ 91274A131_M5x20mm:13
- Mate:146: CNC-006-XAxisMount2:1 ↔ 91263A832-M5x10mm-Countersink:22
- Mate:147: CNC-006-XAxisMount2:1 ↔ 91263A832-M5x10mm-Countersink:23
- Mate:148: CNC-006-XAxisMount2:1 ↔ 91263A832-M5x10mm-Countersink:24
- Mate:149: CNC-006-XAxisMount2:1 ↔ 91263A832-M5x10mm-Countersink:21
- Flush:78: CNC-006-XAxisMount2:1 ↔ 91263A832-M5x10mm-Countersink:21
- Flush:79: CNC-006-XAxisMount2:1 ↔ 91263A832-M5x10mm-Countersink:23
- Flush:80: 91263A832-M5x10mm-Countersink:22 ↔ 91263A832-M5x10mm-Countersink:23
- Flush:81: CNC-006-XAxisMount2:1 ↔ 91263A832-M5x10mm-Countersink:24
- Mate:150: CNC-006-XAxisMount2:1 ↔ 91263A832-M5x10mm-Countersink:25
- Mate:151: CNC-006-XAxisMount2:1 ↔ 91263A832-M5x10mm-Countersink:27
- Mate:152: CNC-006-XAxisMount2:1 ↔ 91263A832-M5x10mm-Countersink:28
- Mate:153: CNC-006-XAxisMount2:1 ↔ 91263A832-M5x10mm-Countersink:26
- Flush:82: CNC-006-XAxisMount2:1 ↔ 91263A832-M5x10mm-Countersink:27
- Flush:83: CNC-006-XAxisMount2:1 ↔ 91263A832-M5x10mm-Countersink:26
- Flush:84: CNC-006-XAxisMount2:1 ↔ 91263A832-M5x10mm-Countersink:28
- Flush:85: CNC-006-XAxisMount2:1 ↔ 91263A832-M5x10mm-Countersink:25
- Mate:154: CNC-006-XAxisMount2:1 ↔ 91263A832-M5x10mm-Countersink:31
- Mate:155: CNC-006-XAxisMount2:1 ↔ 91263A832-M5x10mm-Countersink:30
- Mate:156: CNC-006-XAxisMount2:1 ↔ 91263A832-M5x10mm-Countersink:29
- Mate:157: CNC-006-XAxisMount2:1 ↔ 91263A832-M5x10mm-Countersink:32
- Flush:86: CNC-006-XAxisMount2:1 ↔ 91263A832-M5x10mm-Countersink:32
- Flush:87: CNC-006-XAxisMount2:1 ↔ 91263A832-M5x10mm-Countersink:29
- Flush:88: 91263A832-M5x10mm-Countersink:29 ↔ 91263A832-M5x10mm-Countersink:31
- Flush:89: 91263A832-M5x10mm-Countersink:30 ↔ 91263A832-M5x10mm-Countersink:31
- Mate:158: CNC-006-XAxisMount2:1 ↔ 91263A832-M5x10mm-Countersink:35
- Mate:159: CNC-006-XAxisMount2:1 ↔ 91263A832-M5x10mm-Countersink:33
- Mate:160: CNC-006-XAxisMount2:1 ↔ 91263A832-M5x10mm-Countersink:34
- Mate:161: CNC-006-XAxisMount2:1 ↔ 91263A832-M5x10mm-Countersink:36
- Flush:90: CNC-006-XAxisMount2:1 ↔ 91263A832-M5x10mm-Countersink:36
- Flush:91: CNC-006-XAxisMount2:1 ↔ 91263A832-M5x10mm-Countersink:34
- Flush:92: CNC-006-XAxisMount2:1 ↔ 91263A832-M5x10mm-Countersink:35
- Flush:93: CNC-006-XAxisMount2:1 ↔ 91263A832-M5x10mm-Countersink:33
- Mate:162: CNC-006-XAxisMount2:1 ↔ 91263A832-M5x10mm-Countersink:38
- Mate:163: CNC-006-XAxisMount2:1 ↔ 91263A832-M5x10mm-Countersink:39
- Mate:164: CNC-006-XAxisMount2:1 ↔ 91263A832-M5x10mm-Countersink:37
- Mate:165: CNC-006-XAxisMount2:1 ↔ 91263A832-M5x10mm-Countersink:40
- Flush:94: CNC-006-XAxisMount2:1 ↔ 91263A832-M5x10mm-Countersink:40
- Flush:95: CNC-006-XAxisMount2:1 ↔ 91263A832-M5x10mm-Countersink:37
- Flush:96: CNC-006-XAxisMount2:1 ↔ 91263A832-M5x10mm-Countersink:38
- Flush:97: CNC-006-XAxisMount2:1 ↔ 91263A832-M5x10mm-Countersink:39
- Mate:166: CNC-005-XAxisMount1:1 ↔ CNC-006-XAxisMount2:1
- Mate:167: CNC-006-XAxisMount2:1 ↔ 92095A495-M8-18mm-ButtonHead:1
- Mate:168: CNC-006-XAxisMount2:1 ↔ 92095A495-M8-18mm-ButtonHead:2
- Mate:169: CNC-006-XAxisMount2:1 ↔ 92095A495-M8-18mm-ButtonHead:3
- Mate:170: CNC-006-XAxisMount2:1 ↔ 92095A495-M8-18mm-ButtonHead:3
- Flush:98: 92095A495-M8-18mm-ButtonHead:1 ↔ 92095A495-M8-18mm-ButtonHead:3
- Flush:99: 92095A495-M8-18mm-ButtonHead:1 ↔ 92095A495-M8-18mm-ButtonHead:2
- Mate:171: CNC-006-XAxisMount2:1 ↔ 92095A495-M8-18mm-ButtonHead:8
- Flush:100: 92095A495-M8-18mm-ButtonHead:3 ↔ 92095A495-M8-18mm-ButtonHead:8
- Mate:172: CNC-006-XAxisMount2:1 ↔ 92095A495-M8-18mm-ButtonHead:11
- Mate:173: CNC-006-XAxisMount2:1 ↔ 92095A495-M8-18mm-ButtonHead:12
- Flush:101: 92095A495-M8-18mm-ButtonHead:11 ↔ 92095A495-M8-18mm-ButtonHead:12
- Flush:102: 92095A495-M8-18mm-ButtonHead:1 ↔ 92095A495-M8-18mm-ButtonHead:11
- Mate:174: CNC-006-XAxisMount2:1 ↔ 92095A495-M8-18mm-ButtonHead:9
- Mate:175: CNC-006-XAxisMount2:1 ↔ 92095A495-M8-18mm-ButtonHead:10
- Flush:103: 92095A495-M8-18mm-ButtonHead:9 ↔ 92095A495-M8-18mm-ButtonHead:10
- Flush:104: 92095A495-M8-18mm-ButtonHead:2 ↔ 92095A495-M8-18mm-ButtonHead:9
- Mate:176: 92095A495-M8-18mm-ButtonHead:1 ↔ 94645A210-M8-NylockNut:1
- Mate:177: CNC-005-XAxisMount1:1 ↔ 94645A210-M8-NylockNut:1
- Mate:178: 92095A495-M8-18mm-ButtonHead:2 ↔ 94645A210-M8-NylockNut:2
- Mate:179: CNC-005-XAxisMount1:1 ↔ 94645A210-M8-NylockNut:2
- Mate:180: 92095A495-M8-18mm-ButtonHead:3 ↔ 94645A210-M8-NylockNut:3
- Mate:181: CNC-005-XAxisMount1:1 ↔ 94645A210-M8-NylockNut:3
- Mate:182: 92095A495-M8-18mm-ButtonHead:8 ↔ 94645A210-M8-NylockNut:4
- Mate:183: CNC-005-XAxisMount1:1 ↔ 94645A210-M8-NylockNut:4
- Mate:184: 92095A495-M8-18mm-ButtonHead:11 ↔ 94645A210-M8-NylockNut:5
- Mate:185: 92095A495-M8-18mm-ButtonHead:12 ↔ 94645A210-M8-NylockNut:6
- Mate:186: CNC-005-XAxisMount1:1 ↔ 94645A210-M8-NylockNut:6
- Mate:187: CNC-005-XAxisMount1:1 ↔ 94645A210-M8-NylockNut:5
- Mate:188: 92095A495-M8-18mm-ButtonHead:9 ↔ 94645A210-M8-NylockNut:7
- Mate:189: 92095A495-M8-18mm-ButtonHead:10 ↔ 94645A210-M8-NylockNut:8
- Mate:190: CNC-005-XAxisMount1:1 ↔ 94645A210-M8-NylockNut:8
- Mate:191: CNC-005-XAxisMount1:1 ↔ 94645A210-M8-NylockNut:7
- Mate:192: HGR20R-LinearRail500mm:4 ↔ 20x40x500mm-Extrusion2:1
- Flush:106: HGR20R-LinearRail500mm:4 ↔ 20x40x500mm-Extrusion2:1
- Flush:107: HGR20R-LinearRail500mm:4 ↔ 20x40x500mm-Extrusion2:1
- Flush:108: 20x40x500mm-Extrusion2:1 ↔ 20x40x500mm-Extrusion2:2
- Mate:193: 20x40x500mm-Extrusion2:1 ↔ 20x40x500mm-Extrusion2:2
- Flush:109: 20x40x500mm-Extrusion2:1 ↔ 20x40x500mm-Extrusion2:2
- Flush:110: 20x40x500mm-Extrusion2:2 ↔ 20x40x500mm-Extrusion2:3
- Flush:111: 20x40x500mm-Extrusion2:2 ↔ 20x40x500mm-Extrusion2:3
- Mate:194: 20x40x500mm-Extrusion2:2 ↔ 20x40x500mm-Extrusion2:3
- Flush:112: 20x40x500mm-Extrusion2:3 ↔ 20x20x500mm_Extrusion:1
- Flush:113: 20x40x500mm-Extrusion2:3 ↔ 20x20x500mm_Extrusion:1
- Mate:195: 20x40x500mm-Extrusion2:3 ↔ 20x20x500mm_Extrusion:1
